# Autodesk Inventor assembly: MIRleft中間ユニット
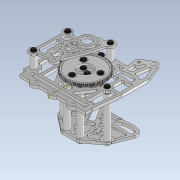
[picture p0: Inventor's stored thumbnail of the model, 180x180]
Saved by Autodesk Inventor 2020.2 (Build 242310000, 310)
## iProperties
Created: 2020-03-12
Part Number: MIRleft中間ユニット
Document SubType Name: Assembly
Designer: aoyama
Mass: 89.3015 g
Surface Area: 374.706 cm^2
Volume: 27.4376 cm^3
Density: 3.25472 g/cm^3
Author: aoyam
## Documents named in this file (30)
- C:\Users\aoyam\Desktop\SRDC_local\Inventor\二年機\Geminiβ\脚\中間ユニット\MIR達\MIRleft中間ユニット.iam
- C:\Users\aoyam\Desktop\SRDC_local\Inventor\二年機\Geminiβ\汎用部品\MIR達\MIRleftワッシャD7d3m0.5.ipt
- C:\Users\aoyam\Desktop\SRDC_local\Inventor\二年機\Geminiβ\脚\中間ユニット\MIR達\MIRleft中間ギア抑え.ipt
- C:\Users\aoyam\Desktop\SRDC_local\Inventor\二年機\Geminiβ\汎用部品\MIR達\MIRleftベアリングd4D8B3F.ipt
- C:\Users\aoyam\Desktop\SRDC_local\Inventor\二年機\Geminiβ\汎用部品\MIR達\MIRleftワッシャD7d4m0.5.ipt
- C:\Users\aoyam\Desktop\SRDC_local\Inventor\二年機\Geminiβ\汎用部品\MIR達\MIRleftｍ2歯数9ギアd3.99.ipt
- C:\Users\aoyam\Desktop\SRDC_local\Inventor\二年機\Geminiβ\汎用部品\MIR達\MIRleftｍ0.5歯数80ギアd15.ipt
- C:\Users\aoyam\Desktop\SRDC_local\Inventor\二年機\Geminiβ\脚\中間ユニット\MIR達\MIRleft脚中間フレームカム.ipt
- C:\Users\aoyam\Desktop\SRDC_local\Inventor\二年機\Geminiβ\汎用部品\MIR達\MIRleftベアリングd15D21B4.ipt
- C:\Users\aoyam\Desktop\SRDC_local\Inventor\二年機\Geminiβ\脚\中間ユニット\MIR達\MIRleft脚中間フレームカム3.ipt
- C:\Users\aoyam\Desktop\SRDC_local\Inventor\二年機\Geminiβ\脚\中間ユニット\MIR達\MIRleft中間フレーム内側.ipt
- C:\Users\aoyam\Desktop\SRDC_local\Inventor\二年機\Geminiβ\汎用部品\MIR達\MIRleftネジ超極低頭M3L8.ipt
- C:\Users\aoyam\Desktop\SRDC_local\Inventor\二年機\Geminiβ\脚\中間ユニット\MIR達\MIRleftモーターマウント.ipt
- C:\Users\aoyam\Desktop\SRDC_local\Inventor\二年機\Geminiβ\汎用部品\MIR達\MIRleftネジボタンM3L4.ipt
- C:\Users\aoyam\Desktop\SRDC_local\Inventor\二年機\Geminiβ\汎用部品\MIR達\MIRleftネジボタンM3L8.ipt
- C:\Users\aoyam\Desktop\SRDC_local\Inventor\二年機\Geminiβ\汎用部品\MIR達\MIRleftスペーサーM3L45アルミ.ipt
- C:\Users\aoyam\Desktop\SRDC_local\Inventor\二年機\Geminiβ\汎用部品\MIR達\MIRleftネジボタンM3L6.ipt
- C:\Users\aoyam\Desktop\SRDC_local\Inventor\二年機\Geminiβ\脚\中間ユニット\MIR達\MIRleft脚中間フレームカム2.ipt
- C:\Users\aoyam\Desktop\SRDC_local\Inventor\二年機\Geminiβ\汎用部品\MIR達\MIRleftネジボタンM3L15.ipt
- C:\Users\aoyam\Desktop\SRDC_local\Inventor\二年機\Geminiβ\汎用部品\MIR達\MIRleftスペーサーM3L15アルミ.ipt
- C:\Users\aoyam\Desktop\SRDC_local\Inventor\二年機\Geminiβ\汎用部品\MIR達\MIRleftスペーサーM3L20アルミ.ipt
- C:\Users\aoyam\Desktop\SRDC_local\Inventor\二年機\Geminiβ\汎用部品\MIR達\MIRleftネジボタンM3L10.ipt
- C:\Users\aoyam\Desktop\SRDC_local\Inventor\二年機\Geminiβ\汎用部品\MIR達\MIRleftスペーサー中空M3L8アルミ.ipt
- C:\Users\aoyam\Desktop\SRDC_local\Inventor\二年機\Geminiβ\脚\中間ユニット\脚中間フレーム外側.ipt
- C:\Users\aoyam\Desktop\SRDC_local\Inventor\二年機\Geminiβ\汎用部品\平行ピンD4L18.ipt
- C:\Users\aoyam\Desktop\SRDC_local\Inventor\二年機\Geminiβ\汎用部品\ネジボタンM3L14.ipt
- C:\Users\aoyam\Desktop\SRDC_local\Inventor\二年機\Geminiβ\汎用部品\スペーサー中空M3L15アルミ.ipt
- C:\Users\aoyam\Desktop\SRDC_local\Inventor\二年機\Geminiβ\汎用部品\ネジボタンM3L18.ipt
- C:\Users\aoyam\Desktop\SRDC_local\Inventor\二年機\Geminiβ\汎用部品\ワッシャD6d3m0.5.ipt
- C:\Users\aoyam\Desktop\SRDC_local\Inventor\二年機\Geminiβ\汎用部品\ネジ超低頭M3L8.ipt
## Components (50 placed, 29 different names)
1. MIRleft中間ギア抑え:1 — 挿入:5, メイト:15, 挿入:84, 挿入:85
2. MIRleftベアリングd4D8B3F:1 — 挿入:5, 挿入:6
3. MIRleftワッシャD7d4m0.5:1 — 挿入:6, 挿入:7
4. MIRleftｍ2歯数9ギアd3.99:1 — 挿入:7, メイト:3, メイト:26, メイト:11
5. MIRleftｍ0.5歯数80ギアd15:1 — 挿入:153, 挿入:11, 挿入:47, 挿入:154, 挿入:50
6. MIRleft脚中間フレームカム:1 — メイト:10, 挿入:10, 挿入:77, メイト:11, メイト:12
7. MIRleftベアリングd15D21B4:1 — メイト:3, 挿入:28, 挿入:79
8. MIRleft脚中間フレームカム3:1 — 挿入:153, メイト:10, 挿入:11, 挿入:10, 挿入:58, 挿入:59, 挿入:60
9. MIRleft中間フレーム内側:1 — メイト:15, 挿入:28, フラッシュ:3, メイト:22, 挿入:64, 挿入:65, 挿入:75, 挿入:149, 挿入:148, 挿入:89, 挿入:175, 挿入:139, 挿入:164, 挿入:170, 挿入:181, 挿入:61, 挿入:62, 挿入:74, 挿入:77
10. MIRleftモーターマウント:1 — 挿入:134, 挿入:140, 挿入:63, 挿入:64, 挿入:70, 挿入:71
11. MIRleftネジボタンM3L4:1 — 挿入:47
12. MIRleftネジボタンM3L4:2 — 挿入:154
13. MIRleftネジボタンM3L4:3 — 挿入:50
14. MIRleftネジボタンM3L8:3 — 挿入:134
15. MIRleftスペーサーM3L45アルミ:1 — メイト:22, 挿入:52
16. MIRleftネジ超極低頭M3L8:4 — 挿入:64
17. MIRleftネジ超極低頭M3L8:5 — 挿入:65
18. MIRleftネジボタンM3L6:1 — 挿入:75
19. MIRleft脚中間フレームカム2:1 — 挿入:79, メイト:26, 挿入:77, メイト:12
20. MIRleftスペーサーM3L45アルミ:2 — 挿入:149
21. MIRleftスペーサーM3L45アルミ:3 — 挿入:148
22. MIRleftワッシャD7d3m0.5:2 — 挿入:84
23. MIRleftワッシャD7d3m0.5:3 — 挿入:85, 挿入:86
24. MIRleftネジボタンM3L15:1 — 挿入:86
25. MIRleftネジボタンM3L8:4 — 挿入:89
26. MIRleftスペーサーM3L45アルミ:4 — 挿入:69, 挿入:78
27. MIRleftネジボタンM3L8:5 — 挿入:175
28. MIRleftスペーサーM3L15アルミ:1 — 挿入:140, 挿入:139
29. MIRleftスペーサーM3L20アルミ:1 — 挿入:164, 挿入:171
30. MIRleftネジボタンM3L6:2 — 挿入:170
31. MIRleftネジボタンM3L10:1 — 挿入:171
32. MIRleftスペーサー中空M3L8アルミ:1 — 挿入:181
33. 脚中間フレーム外側:1 — 挿入:52, 挿入:69, 挿入:79, 挿入:80, 挿入:81, 挿入:82
34. 平行ピンD4L18:1 — 挿入:58
35. ネジボタンM3L14:1 — 挿入:60
36. ネジボタンM3L14:2 — 挿入:59
37. スペーサー中空M3L15アルミ:1 — 挿入:61, 挿入:64
38. スペーサー中空M3L15アルミ:2 — 挿入:62, 挿入:63
39. ネジボタンM3L18:1 — 挿入:70
40. ネジボタンM3L18:2 — 挿入:71
41. ワッシャD6d3m0.5:1 — 挿入:72, 挿入:73
42. ワッシャD6d3m0.5:2 — 挿入:72, 挿入:74
43. ワッシャD6d3m0.5:3 — 挿入:73
44. ワッシャD6d3m0.5:4 — 挿入:75, 挿入:76
45. ワッシャD6d3m0.5:5 — 挿入:75, 挿入:77
46. ワッシャD6d3m0.5:6 — 挿入:76, 挿入:78
47. ネジ超低頭M3L8:1 — 挿入:79
48. ネジ超低頭M3L8:2 — 挿入:80
49. ネジ超低頭M3L8:3 — 挿入:81
50. ネジ超低頭M3L8:4 — 挿入:82
## Relationships (59: Insert 51, Mate 7, Flush 1)
- 挿入:5 [Insert]: MIRleft中間ギア抑え:1 ↔ MIRleftベアリングd4D8B3F:1
- 挿入:6 [Insert]: MIRleftベアリングd4D8B3F:1 ↔ MIRleftワッシャD7d4m0.5:1
- 挿入:7 [Insert]: MIRleftワッシャD7d4m0.5:1 ↔ MIRleftｍ2歯数9ギアd3.99:1
- メイト:3 [Mate]: MIRleftｍ2歯数9ギアd3.99:1 ↔ MIRleftベアリングd15D21B4:1
- 挿入:153 [Insert]: MIRleftｍ0.5歯数80ギアd15:1 ↔ MIRleft脚中間フレームカム3:1
- メイト:10 [Mate]: MIRleft脚中間フレームカム:1 ↔ MIRleft脚中間フレームカム3:1
- 挿入:11 [Insert]: MIRleftｍ0.5歯数80ギアd15:1 ↔ MIRleft脚中間フレームカム3:1
- 挿入:10 [Insert]: MIRleft脚中間フレームカム:1 ↔ MIRleft脚中間フレームカム3:1
- メイト:15 [Mate]: MIRleft中間ギア抑え:1 ↔ MIRleft中間フレーム内側:1
- 挿入:28 [Insert]: MIRleftベアリングd15D21B4:1 ↔ MIRleft中間フレーム内側:1
- 挿入:47 [Insert]: MIRleftｍ0.5歯数80ギアd15:1 ↔ MIRleftネジボタンM3L4:1
- 挿入:154 [Insert]: MIRleftｍ0.5歯数80ギアd15:1 ↔ MIRleftネジボタンM3L4:2
- 挿入:50 [Insert]: MIRleftｍ0.5歯数80ギアd15:1 ↔ MIRleftネジボタンM3L4:3
- 挿入:134 [Insert]: MIRleftモーターマウント:1 ↔ MIRleftネジボタンM3L8:3
- フラッシュ:3 [Flush] (-38 mm): MIRleft中間フレーム内側:1
- メイト:22 [Mate]: MIRleft中間フレーム内側:1 ↔ MIRleftスペーサーM3L45アルミ:1
- 挿入:64 [Insert]: MIRleft中間フレーム内側:1 ↔ MIRleftネジ超極低頭M3L8:4
- 挿入:65 [Insert]: MIRleft中間フレーム内側:1 ↔ MIRleftネジ超極低頭M3L8:5
- 挿入:75 [Insert]: MIRleft中間フレーム内側:1 ↔ MIRleftネジボタンM3L6:1
- 挿入:79 [Insert]: MIRleftベアリングd15D21B4:1 ↔ MIRleft脚中間フレームカム2:1
- メイト:26 [Mate]: MIRleftｍ2歯数9ギアd3.99:1 ↔ MIRleft脚中間フレームカム2:1
- 挿入:77 [Insert]: MIRleft脚中間フレームカム:1 ↔ MIRleft脚中間フレームカム2:1
- 挿入:149 [Insert]: MIRleft中間フレーム内側:1 ↔ MIRleftスペーサーM3L45アルミ:2
- 挿入:148 [Insert]: MIRleft中間フレーム内側:1 ↔ MIRleftスペーサーM3L45アルミ:3
- 挿入:84 [Insert]: MIRleft中間ギア抑え:1 ↔ MIRleftワッシャD7d3m0.5:2
- 挿入:85 [Insert]: MIRleft中間ギア抑え:1 ↔ MIRleftワッシャD7d3m0.5:3
- 挿入:86 [Insert] (3 mm): MIRleftワッシャD7d3m0.5:3 ↔ MIRleftネジボタンM3L15:1
- 挿入:89 [Insert]: MIRleft中間フレーム内側:1 ↔ MIRleftネジボタンM3L8:4
- 挿入:175 [Insert]: MIRleft中間フレーム内側:1 ↔ MIRleftネジボタンM3L8:5
- 挿入:140 [Insert]: MIRleftモーターマウント:1 ↔ MIRleftスペーサーM3L15アルミ:1
- 挿入:139 [Insert]: MIRleft中間フレーム内側:1 ↔ MIRleftスペーサーM3L15アルミ:1
- 挿入:164 [Insert]: MIRleft中間フレーム内側:1 ↔ MIRleftスペーサーM3L20アルミ:1
- 挿入:170 [Insert]: MIRleft中間フレーム内側:1 ↔ MIRleftネジボタンM3L6:2
- 挿入:171 [Insert] (5 mm): MIRleftスペーサーM3L20アルミ:1 ↔ MIRleftネジボタンM3L10:1
- 挿入:181 [Insert]: MIRleft中間フレーム内側:1 ↔ MIRleftスペーサー中空M3L8アルミ:1
- 挿入:52 [Insert]: MIRleftスペーサーM3L45アルミ:1 ↔ 脚中間フレーム外側:1
- メイト:11 [Mate]: MIRleftｍ2歯数9ギアd3.99:1 ↔ MIRleft脚中間フレームカム:1
- メイト:12 [Mate]: MIRleft脚中間フレームカム:1 ↔ MIRleft脚中間フレームカム2:1
- 挿入:58 [Insert]: MIRleft脚中間フレームカム3:1 ↔ 平行ピンD4L18:1
- 挿入:59 [Insert]: MIRleft脚中間フレームカム3:1 ↔ ネジボタンM3L14:2
- 挿入:60 [Insert]: MIRleft脚中間フレームカム3:1 ↔ ネジボタンM3L14:1
- 挿入:61 [Insert]: MIRleft中間フレーム内側:1 ↔ スペーサー中空M3L15アルミ:1
- 挿入:62 [Insert]: MIRleft中間フレーム内側:1 ↔ スペーサー中空M3L15アルミ:2
- 挿入:63 [Insert]: MIRleftモーターマウント:1 ↔ スペーサー中空M3L15アルミ:2
- 挿入:64 [Insert]: MIRleftモーターマウント:1 ↔ スペーサー中空M3L15アルミ:1
- 挿入:69 [Insert]: MIRleftスペーサーM3L45アルミ:4 ↔ 脚中間フレーム外側:1
- 挿入:70 [Insert]: MIRleftモーターマウント:1 ↔ ネジボタンM3L18:1
- 挿入:71 [Insert]: MIRleftモーターマウント:1 ↔ ネジボタンM3L18:2
- 挿入:72 [Insert]: ワッシャD6d3m0.5:1 ↔ ワッシャD6d3m0.5:2
- 挿入:73 [Insert]: ワッシャD6d3m0.5:1 ↔ ワッシャD6d3m0.5:3
- 挿入:74 [Insert]: MIRleft中間フレーム内側:1 ↔ ワッシャD6d3m0.5:2
- 挿入:75 [Insert]: ワッシャD6d3m0.5:4 ↔ ワッシャD6d3m0.5:5
- 挿入:76 [Insert]: ワッシャD6d3m0.5:4 ↔ ワッシャD6d3m0.5:6
- 挿入:77 [Insert]: MIRleft中間フレーム内側:1 ↔ ワッシャD6d3m0.5:5
- 挿入:78 [Insert]: MIRleftスペーサーM3L45アルミ:4 ↔ ワッシャD6d3m0.5:6
- 挿入:79 [Insert]: 脚中間フレーム外側:1 ↔ ネジ超低頭M3L8:1
- 挿入:80 [Insert]: 脚中間フレーム外側:1 ↔ ネジ超低頭M3L8:2
- 挿入:81 [Insert]: 脚中間フレーム外側:1 ↔ ネジ超低頭M3L8:3
- 挿入:82 [Insert]: 脚中間フレーム外側:1 ↔ ネジ超低頭M3L8:4
